# Autodesk Inventor assembly: FrontLink
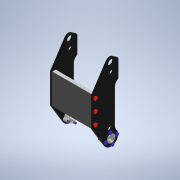
[picture p0: Inventor's stored thumbnail of the model, 180x180]
Saved by Autodesk Inventor 2020 (Build 240168000, 168)
## iProperties
Created: 2022-06-14
Part Number: FrontLink
Document SubType Name: Assembly
Designer: Masato Kubotera
Author: Masato Kubotera
## Documents named in this file (8)
- C:\Users\MasatoKubotera\Documents\Inventor\SUSTAINA-OP\LowerBody\Link\FrontLink.iam
- C:\Users\MasatoKubotera\Documents\Inventor\SUSTAINA-OP\LowerBody\Link\FrontLink_diagonal.ipt
- C:\Users\MasatoKubotera\Documents\Inventor\SUSTAINA-OP\LowerBody\Link\FrontLink_diagonal_cover_sheet.ipt
- C:\Users\MasatoKubotera\Documents\Inventor\SUSTAINA-OP\LowerBody\Link\FrontLink_frame.ipt
- C:\Users\MasatoKubotera\Documents\Inventor\SUSTAINA-OP\ReadyMade\Washer\WSSS-12-10-8.ipt
- C:\Users\MasatoKubotera\Documents\Inventor\SUSTAINA-OP\LowerBody\Knee\Knee_clamp.ipt
- C:\Users\MasatoKubotera\Documents\Inventor\SUSTAINA-OP\ReadyMade\Screw\M2_6-10.ipt
- C:\Users\MasatoKubotera\Documents\Inventor\SUSTAINA-OP\ReadyMade\Screw\M3-6.ipt
## Components (22 placed, 7 different names)
1. FrontLink_diagonal:1 — フラッシュ:1, フラッシュ:2, フラッシュ:3, 挿入:1, 挿入:2, 挿入:3, 挿入:4, 挿入:5, 挿入:6, フラッシュ:4, フラッシュ:5, メイト:1
2. FrontLink_diagonal_cover_sheet:1 — フラッシュ:4, フラッシュ:5, メイト:1
3. FrontLink_frame:1 — 挿入:1, 挿入:2, 挿入:3, 挿入:9, 挿入:10, 挿入:11, 挿入:12, 挿入:17, 挿入:18, 挿入:19, 挿入:20, 挿入:25, 挿入:26, 挿入:27
4. FrontLink_frame:2 — 挿入:4, 挿入:5, 挿入:6, 挿入:13, 挿入:14, 挿入:15, 挿入:16, 挿入:21, 挿入:22, 挿入:23, 挿入:24, 挿入:28, 挿入:29, 挿入:30
5. Knee_clamp:1 — 挿入:7, 挿入:9, 挿入:10, 挿入:11, 挿入:12
6. Knee_clamp:2 — 挿入:8, 挿入:13, 挿入:14, 挿入:15, 挿入:16
7. WSSS-12-10-8:1 — 挿入:7
8. WSSS-12-10-8:2 — 挿入:8
9. M2_6-10:1 — 挿入:17
10. M2_6-10:2 — 挿入:18
11. M2_6-10:3 — 挿入:19
12. M2_6-10:4 — 挿入:20
13. M2_6-10:5 — 挿入:21
14. M2_6-10:6 — 挿入:22
15. M2_6-10:7 — 挿入:23
16. M2_6-10:8 — 挿入:24
17. M3-6:1 — 挿入:25
18. M3-6:2 — 挿入:26
19. M3-6:3 — 挿入:27
20. M3-6:4 — 挿入:28
21. M3-6:5 — 挿入:29
22. M3-6:6 — 挿入:30
## Relationships (36: Insert 30, Flush 5, Mate 1)
- フラッシュ:1 [Flush]: FrontLink_diagonal:1
- フラッシュ:2 [Flush]: FrontLink_diagonal:1
- フラッシュ:3 [Flush]: FrontLink_diagonal:1
- 挿入:1 [Insert]: FrontLink_diagonal:1 ↔ FrontLink_frame:1
- 挿入:2 [Insert]: FrontLink_diagonal:1 ↔ FrontLink_frame:1
- 挿入:3 [Insert]: FrontLink_diagonal:1 ↔ FrontLink_frame:1
- 挿入:4 [Insert]: FrontLink_diagonal:1 ↔ FrontLink_frame:2
- 挿入:5 [Insert]: FrontLink_diagonal:1 ↔ FrontLink_frame:2
- 挿入:6 [Insert]: FrontLink_diagonal:1 ↔ FrontLink_frame:2
- フラッシュ:4 [Flush]: FrontLink_diagonal:1 ↔ FrontLink_diagonal_cover_sheet:1
- フラッシュ:5 [Flush]: FrontLink_diagonal:1 ↔ FrontLink_diagonal_cover_sheet:1
- メイト:1 [Mate]: FrontLink_diagonal:1 ↔ FrontLink_diagonal_cover_sheet:1
- 挿入:7 [Insert]: Knee_clamp:1 ↔ WSSS-12-10-8:1
- 挿入:8 [Insert]: Knee_clamp:2 ↔ WSSS-12-10-8:2
- 挿入:9 [Insert]: FrontLink_frame:1 ↔ Knee_clamp:1
- 挿入:10 [Insert]: FrontLink_frame:1 ↔ Knee_clamp:1
- 挿入:11 [Insert]: FrontLink_frame:1 ↔ Knee_clamp:1
- 挿入:12 [Insert]: FrontLink_frame:1 ↔ Knee_clamp:1
- 挿入:13 [Insert]: FrontLink_frame:2 ↔ Knee_clamp:2
- 挿入:14 [Insert]: FrontLink_frame:2 ↔ Knee_clamp:2
- 挿入:15 [Insert]: FrontLink_frame:2 ↔ Knee_clamp:2
- 挿入:16 [Insert]: FrontLink_frame:2 ↔ Knee_clamp:2
- 挿入:17 [Insert]: FrontLink_frame:1 ↔ M2_6-10:1
- 挿入:18 [Insert]: FrontLink_frame:1 ↔ M2_6-10:2
- 挿入:19 [Insert]: FrontLink_frame:1 ↔ M2_6-10:3
- 挿入:20 [Insert]: FrontLink_frame:1 ↔ M2_6-10:4
- 挿入:21 [Insert]: FrontLink_frame:2 ↔ M2_6-10:5
- 挿入:22 [Insert]: FrontLink_frame:2 ↔ M2_6-10:6
- 挿入:23 [Insert]: FrontLink_frame:2 ↔ M2_6-10:7
- 挿入:24 [Insert]: FrontLink_frame:2 ↔ M2_6-10:8
- 挿入:25 [Insert]: FrontLink_frame:1 ↔ M3-6:1
- 挿入:26 [Insert]: FrontLink_frame:1 ↔ M3-6:2
- 挿入:27 [Insert]: FrontLink_frame:1 ↔ M3-6:3
- 挿入:28 [Insert]: FrontLink_frame:2 ↔ M3-6:4
- 挿入:29 [Insert]: FrontLink_frame:2 ↔ M3-6:5
- 挿入:30 [Insert]: FrontLink_frame:2 ↔ M3-6:6
